# Autodesk Inventor assembly: s-assy-spacer4
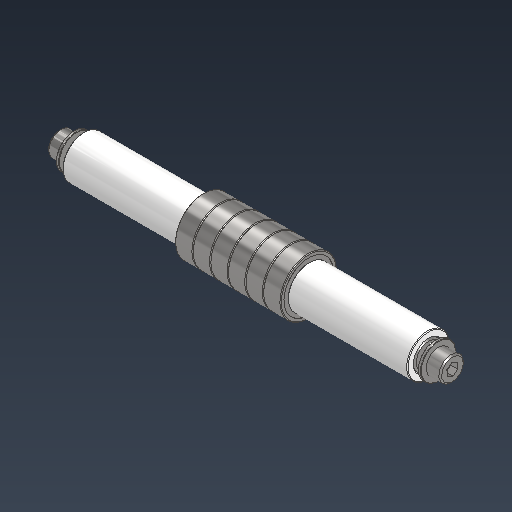
[picture p0: Inventor's stored thumbnail of the model, 512x512]
Saved by Autodesk Inventor 2021 (Build 250183000, 183)
## iProperties
Created: 2021-07-17
Part Number: s-assy-spacer4
Document SubType Name: Assembly
Designer: yuta0
Author: yuta0
## Documents named in this file (6)
- C:\Users\yuta0\Documents\GitHub\catchrobo_hardware\assy-robot\s-assy-spacer4.iam
- C:\Users\yuta0\Documents\GitHub\catchrobo_hardware\assy-robot\base17.ipt
- C:\Users\yuta0\Documents\GitHub\catchrobo_hardware\assy-robot\B688ZZ.ipt
- C:\Users\yuta0\Documents\GitHub\catchrobo_hardware\assy-robot\SFHRW8-98-M4-N4.ipt
- C:\Users\yuta0\Documents\GitHub\catchrobo_hardware\assy-robot\CB4-10.ipt
- C:\Users\yuta0\Documents\GitHub\catchrobo_hardware\assy-robot\WSJ-STN-M4.ipt
## Components (13 placed, 5 different names)
1. spacer2:1 — メイト:13, メイト:18, フラッシュ:1
2. spacer2:2 — メイト:15, メイト:17
3. SFHRW8-98-M4-N4:1 — メイト:18, フラッシュ:1, メイト:19, メイト:20, メイト:21, メイト:24, メイト:27
4. CB4-10:1 — メイト:20, メイト:22, メイト:23
5. WSJ-STN-M4:1 — メイト:22, メイト:23, メイト:24
6. CB4-10:2 — メイト:21, メイト:25, メイト:26
7. WSJ-STN-M4:2 — メイト:25, メイト:26, メイト:27
8. B688ZZ:2 — メイト:13, メイト:19
9. B688ZZ:3
10. B688ZZ:4
11. B688ZZ:5
12. B688ZZ:6 — メイト:17
13. B688ZZ:7 — メイト:15
## Component patterns: (6 elements, first: B688ZZ:2)
## Relationships (14: Mate 13, Flush 1)
- メイト:13 [Mate]: spacer2:1 ↔ B688ZZ:2
- メイト:15 [Mate]: spacer2:2 ↔ B688ZZ:7
- メイト:17 [Mate]: spacer2:2 ↔ B688ZZ:6
- メイト:18 [Mate]: spacer2:1 ↔ SFHRW8-98-M4-N4:1
- フラッシュ:1 [Flush]: spacer2:1 ↔ SFHRW8-98-M4-N4:1
- メイト:19 [Mate]: SFHRW8-98-M4-N4:1 ↔ B688ZZ:2
- メイト:20 [Mate]: SFHRW8-98-M4-N4:1 ↔ CB4-10:1
- メイト:21 [Mate]: SFHRW8-98-M4-N4:1 ↔ CB4-10:2
- メイト:22 [Mate]: CB4-10:1 ↔ WSJ-STN-M4:1
- メイト:23 [Mate]: CB4-10:1 ↔ WSJ-STN-M4:1
- メイト:24 [Mate] (2 mm): SFHRW8-98-M4-N4:1 ↔ WSJ-STN-M4:1
- メイト:25 [Mate]: CB4-10:2 ↔ WSJ-STN-M4:2
- メイト:26 [Mate]: CB4-10:2 ↔ WSJ-STN-M4:2
- メイト:27 [Mate] (2 mm): SFHRW8-98-M4-N4:1 ↔ WSJ-STN-M4:2
